# Autodesk Inventor assembly: Mechanism Platform
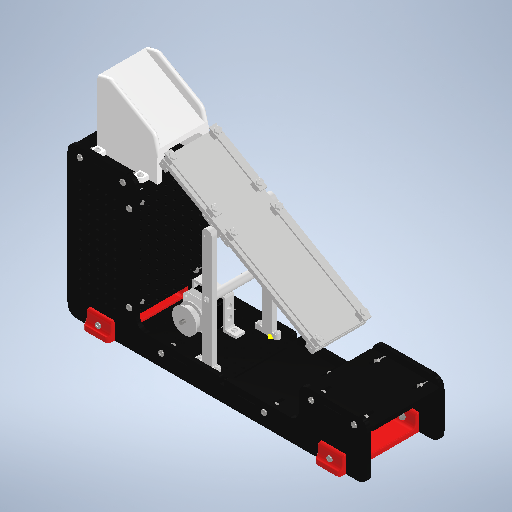
[picture p0: Inventor's stored thumbnail of the model, 512x512]
Saved by Autodesk Inventor 2025 (Build 290162000, 162)
## iProperties
Manager: Yassa Basem
Company: ENG 1P13
Created: 2024-06-07
Part Number: Mechanism Platform
Document SubType Name: Assembly
Designer: Alex Forbes
Checked By: Yassa Basem
Engineer: Alex Forbes
Author: A 1P13 IAI
Title: Mechanism Platform
## Documents named in this file (21)
- C:\Users\liaco\OneDrive\Documents\Graphics Labs\1P13 CAD Models\Design 2\Platform Assembly\1. Platform\Mechanism Platform.iam
- C:\Users\liaco\OneDrive\Documents\Graphics Labs\1P13 CAD Models\Design 2\Platform Assembly\1. Platform\Mounting Base Middle.ipt
- C:\Users\liaco\OneDrive\Documents\Graphics Labs\1P13 CAD Models\Design 2\Platform Assembly\1. Platform\Mounting Base Side.ipt
- C:\Users\liaco\OneDrive\Documents\Graphics Labs\1P13 CAD Models\Design 2\Platform Assembly\1. Platform\ANSI B 18.2.4.1 M - M4 x 0.7Style 1.ipt
- C:\Users\liaco\OneDrive\Documents\Graphics Labs\1P13 CAD Models\Design 2\Platform Assembly\1. Platform\Mounting Base Bottom.ipt
- C:\Users\liaco\OneDrive\Documents\Graphics Labs\1P13 CAD Models\Design 2\Platform Assembly\1. Platform\ANSI B18.6.7M - M4x0.7 x 20(4).ipt
- C:\Users\liaco\OneDrive\Documents\Graphics Labs\1P13 CAD Models\Design 2\Platform Assembly\1. Platform\Mounting Feet.ipt
- C:\Users\liaco\OneDrive\Documents\Graphics Labs\1P13 CAD Models\Design 2\Platform Assembly\1. Platform\Mounting Side Wall.ipt
- C:\Users\liaco\OneDrive\Documents\Graphics Labs\1P13 CAD Models\Design 2\Platform Assembly\1. Platform\Mounting Base Top.ipt
- C:\Users\liaco\OneDrive\Documents\Graphics Labs\1P13 CAD Models\Design 2\Top Ramp.ipt
- C:\Users\liaco\OneDrive\Documents\Graphics Labs\1P13 CAD Models\Design 2\Slide Strut.ipt
- C:\Users\liaco\OneDrive\Documents\Graphics Labs\1P13 CAD Models\Design 2\Slide Axle.ipt
- C:\Users\liaco\OneDrive\Documents\Graphics Labs\1P13 CAD Models\Design 2\Rotary Actuator Assembly\4. Rotary Actuator\Stepper Motor NEMA 17.iam
- C:\Users\liaco\OneDrive\Documents\Graphics Labs\1P13 CAD Models\Design 2\Rotary Actuator Mount.ipt
- C:\Users\liaco\OneDrive\Documents\Graphics Labs\1P13 CAD Models\Design 2\Pulley.ipt
- C:\Users\liaco\OneDrive\Documents\Graphics Labs\1P13 CAD Models\Design 2\Slide Assembly V2.iam
- C:\Users\liaco\OneDrive\Documents\Graphics Labs\1P13 CAD Models\Design 2\2. Plate Fasteners\M4 x 16mm Machine Screw.ipt
- C:\Users\liaco\OneDrive\Documents\Graphics Labs\1P13 CAD Models\Design 2\support pole.ipt
- C:\Users\liaco\OneDrive\Documents\Graphics Labs\1P13 CAD Models\Design 2\91251A198_Black-Oxide Alloy Steel Socket Head Screw\91251A198_Black-Oxide Alloy Steel Socket Head Screw.ipt
- C:\Users\liaco\OneDrive\Documents\Graphics Labs\1P13 CAD Models\Design 2\2. Plate Fasteners\M4 Nut.ipt
- C:\Users\liaco\OneDrive\Documents\Graphics Labs\1P13 CAD Models\Design 2\90480A009_Low-Strength Steel Hex Nut\90480A009_Low-Strength Steel Hex Nut.ipt
## Components (95 placed, 20 different names)
1. Top Ramp:1 — Mate:200, Mate:201, Mate:202, Mate:240, Mate:241, Mate:242, Mate:243, Mate:244, Mate:245, Mate:246, Mate:247
2. Slide Axle:1 — Angle:11, Mate:224, Mate:234, Flush:5, Angle:13
3. Stepper Motor NEMA 17:1 [sub-assembly] — Flush:4, Mate:265, Mate:266, Mate:267, Flush:6, Mate:272
4. Rotary Actuator Mount:1 — Mate:221, Flush:4, Mate:222, Mate:223, Mate:248, Mate:249, Mate:250, Mate:251, Mate:265, Mate:266
5. Pulley:1 — Mate:267, Flush:6, Mate:272
6. Slide Assembly V2:1 [sub-assembly] — Mate:224, Mate:235, Angle:12, Mate:273, Mate:274, Mate:275, Mate:276, Mate:277, Mate:278, Mate:279, Mate:280, Mate:281, Mate:282, Mate:283, Mate:284, Mate:285, Mate:286, Mate:287, Mate:288, Mate:300, Mate:303, Mate:304, Mate:306, Mate:311, Mate:312, Mate:313, Mate:314
7. Slide Strut:2 — Mate:227, Mate:234, Mate:235, Mate:236, Mate:237, Mate:252, Mate:253, Mate:258, Mate:259, Mate:260, Mate:262, Flush:5, Mate:268, Mate:271
8. Slide Strut:3 — Mate:231, Mate:238, Mate:239, Mate:254, Mate:255, Mate:256, Mate:257, Mate:263, Mate:264, Mate:269, Mate:270
9. support pole:1 — Mate:260, Mate:262, Mate:263, Mate:264, Angle:14
10. Mounting Side Wall:1 — Insert:1, Angle:1, Insert:2, Mate:1, Mate:2, Mate:3, Mate:4, Flush:1, Flush:2, Mate:5, Angle:3, Mate:6, Mate:7, Mate:8, Mate:9, Mate:50, Mate:51, Mate:52, Mate:53, Mate:109, Mate:110, Mate:111, Mate:129, Mate:130, Mate:131, Mate:133, Mate:134, Mate:135, Mate:145, Mate:146, Mate:147, Mate:149, Mate:150, Mate:151, Mate:157, Mate:158, Mate:159, Mate:169, Mate:170, Mate:171, Mate:173, Mate:174, Mate:175, Angle:13
11. Mounting Side Wall:2 — Mate:4, Flush:1, Flush:2, Mate:117, Mate:118, Mate:119, Mate:121, Mate:122, Mate:123, Mate:125, Mate:126, Mate:127, Mate:137, Mate:138, Mate:139, Mate:141, Mate:142, Mate:143, Mate:153, Mate:154, Mate:155, Mate:161, Mate:162, Mate:163, Mate:165, Mate:166, Mate:167
12. Mounting Base Top:1 — Mate:1, Mate:8, Mate:9, Mate:112, Mate:120, Mate:124, Mate:176, Angle:6, Angle:7, Mate:200, Mate:201, Mate:202
13. Mounting Base Middle:1 — Mate:2, Mate:52, Mate:53, Mate:144, Mate:148, Mate:152, Mate:156, Mate:221, Mate:222, Mate:223, Mate:227, Mate:231, Mate:236, Mate:237, Mate:238, Mate:239, Angle:12
14. Mounting Base Bottom:1 — Mate:3, Mate:50, Mate:51, Mate:160, Mate:164, Mate:168, Mate:172, Angle:4, Angle:5
15. Mounting Base Side:1 — Mate:5, Angle:3, Mate:6, Mate:7, Mate:128, Mate:132, Mate:136, Mate:140
16. Mounting Feet:1 — Insert:1, Angle:1, Angle:2, Mate:177, Mate:178, Mate:179, Mate:180, Mate:181, Mate:182, Mate:183, Mate:184
17. Mounting Feet:2 — Insert:2, Angle:2, Mate:185, Mate:186, Mate:187, Mate:188, Mate:189, Mate:190, Mate:191, Mate:192
18. Cross Recessed Pan Head Machine Screw - Type I - Metric M4x0.7 x 20:1 — Mate:173, Mate:174
19. Hex Nut Metric M4 x 0.7:1 — Mate:175, Mate:176
20. Cross Recessed Pan Head Machine Screw - Type I - Metric M4x0.7 x 20:7 — Mate:129, Mate:130
21. Hex Nut Metric M4 x 0.7:3 — Mate:131, Mate:132
22. Cross Recessed Pan Head Machine Screw - Type I - Metric M4x0.7 x 20:8 — Mate:133, Mate:134
23. Hex Nut Metric M4 x 0.7:5 — Mate:135, Mate:136
24. Cross Recessed Pan Head Machine Screw - Type I - Metric M4x0.7 x 20:5 — Mate:121, Mate:122
25. Hex Nut Metric M4 x 0.7:6 — Mate:123, Mate:124
26. Cross Recessed Pan Head Machine Screw - Type I - Metric M4x0.7 x 20:4 — Mate:117, Mate:118
27. Hex Nut Metric M4 x 0.7:7 — Mate:119, Mate:120
28. Cross Recessed Pan Head Machine Screw - Type I - Metric M4x0.7 x 20:6 — Mate:125, Mate:126
29. Hex Nut Metric M4 x 0.7:8 — Mate:127, Mate:128
30. Cross Recessed Pan Head Machine Screw - Type I - Metric M4x0.7 x 20:3 — Mate:137, Mate:138
31. Hex Nut Metric M4 x 0.7:10 — Mate:139, Mate:140
32. Cross Recessed Pan Head Machine Screw - Type I - Metric M4x0.7 x 20:10 — Mate:145, Mate:146
33. Hex Nut Metric M4 x 0.7:11 — Mate:147, Mate:148
34. Cross Recessed Pan Head Machine Screw - Type I - Metric M4x0.7 x 20:11 — Mate:149, Mate:150
35. Hex Nut Metric M4 x 0.7:13 — Mate:151, Mate:152
36. Cross Recessed Pan Head Machine Screw - Type I - Metric M4x0.7 x 20:9 — Mate:141, Mate:142
37. Hex Nut Metric M4 x 0.7:14 — Mate:143, Mate:144
38. Cross Recessed Pan Head Machine Screw - Type I - Metric M4x0.7 x 20:12 — Mate:153, Mate:154
39. Hex Nut Metric M4 x 0.7:16 — Mate:155, Mate:156
40. Cross Recessed Pan Head Machine Screw - Type I - Metric M4x0.7 x 20:13 — Mate:157, Mate:158
41. Hex Nut Metric M4 x 0.7:17 — Mate:159, Mate:160
42. Cross Recessed Pan Head Machine Screw - Type I - Metric M4x0.7 x 20:16 — Mate:169, Mate:170
43. Hex Nut Metric M4 x 0.7:18 — Mate:171, Mate:172
44. Cross Recessed Pan Head Machine Screw - Type I - Metric M4x0.7 x 20:14 — Mate:161, Mate:162
45. Hex Nut Metric M4 x 0.7:19 — Mate:163, Mate:164
46. Cross Recessed Pan Head Machine Screw - Type I - Metric M4x0.7 x 20:15 — Mate:165, Mate:166
47. Hex Nut Metric M4 x 0.7:20 — Mate:167, Mate:168
48. Cross Recessed Pan Head Machine Screw - Type I - Metric M4x0.7 x 20:2 — Mate:109, Mate:110
49. Hex Nut Metric M4 x 0.7:21 — Mate:111, Mate:112
50. Cross Recessed Pan Head Machine Screw - Type I - Metric M4x0.7 x 20:17 — Mate:177, Mate:178
51. Hex Nut Metric M4 x 0.7:22 — Mate:179, Mate:180, Angle:6
52. Cross Recessed Pan Head Machine Screw - Type I - Metric M4x0.7 x 20:18 — Mate:181, Mate:182
53. Hex Nut Metric M4 x 0.7:23 — Mate:183, Mate:184, Angle:7
54. Cross Recessed Pan Head Machine Screw - Type I - Metric M4x0.7 x 20:19 — Mate:185, Mate:186
55. Hex Nut Metric M4 x 0.7:24 — Mate:187, Mate:188, Angle:5
56. Cross Recessed Pan Head Machine Screw - Type I - Metric M4x0.7 x 20:20 — Mate:189, Mate:190
57. Hex Nut Metric M4 x 0.7:25 — Mate:191, Mate:192, Angle:4
58. 90480A009_Low-Strength Steel Hex Nut:8 — Mate:309, Mate:312
59. 90480A009_Low-Strength Steel Hex Nut:7 — Mate:310, Mate:311
60. 90480A009_Low-Strength Steel Hex Nut:6 — Mate:308, Mate:313
61. 90480A009_Low-Strength Steel Hex Nut:5 — Mate:307, Mate:314
62. 90480A009_Low-Strength Steel Hex Nut:4 — Mate:301, Mate:303
63. 90480A009_Low-Strength Steel Hex Nut:3 — Mate:302, Mate:304
64. 90480A009_Low-Strength Steel Hex Nut:2 — Mate:299, Mate:300
65. 90480A009_Low-Strength Steel Hex Nut:1 — Mate:305, Mate:306
66. M4 Nut:10 — Flush:8, Mate:290
67. M4 Nut:9 — Flush:7, Mate:289
68. M4 Nut:8 — Flush:9, Mate:291
69. M4 Nut:7 — Flush:11, Mate:293
70. M4 Nut:6 — Flush:10, Mate:292
71. M4 Nut:5 — Mate:294, Flush:12
72. M4 Nut:4 — Flush:13, Mate:295
73. M4 Nut:3 — Mate:298, Flush:16
74. M4 Nut:2 — Mate:296, Flush:14
75. M4 Nut:1 — Mate:297, Flush:15
76. 91251A198_Black-Oxide Alloy Steel Socket Head Screw:1 — Mate:273, Mate:277, Mate:299
77. 91251A198_Black-Oxide Alloy Steel Socket Head Screw:2 — Mate:276, Mate:280, Mate:305
78. 91251A198_Black-Oxide Alloy Steel Socket Head Screw:3 — Mate:274, Mate:278, Mate:301
79. 91251A198_Black-Oxide Alloy Steel Socket Head Screw:4 — Mate:275, Mate:279, Mate:302
80. 91251A198_Black-Oxide Alloy Steel Socket Head Screw:5 — Mate:284, Mate:288, Mate:307
81. 91251A198_Black-Oxide Alloy Steel Socket Head Screw:6 — Mate:283, Mate:287, Mate:308
82. 91251A198_Black-Oxide Alloy Steel Socket Head Screw:7 — Mate:282, Mate:286, Mate:309
83. 91251A198_Black-Oxide Alloy Steel Socket Head Screw:8 — Mate:281, Mate:285, Mate:310
84. M4 x 16mm Machine Screw:13 — Mate:269, Mate:270
85. M4 x 16mm Machine Screw:12 — Mate:268, Mate:271
86. M4 x 16mm Machine Screw:10 — Mate:253, Mate:259, Mate:297, Flush:15
87. M4 x 16mm Machine Screw:9 — Mate:254, Mate:257, Flush:13, Mate:295
88. M4 x 16mm Machine Screw:8 — Mate:252, Mate:258, Mate:298, Flush:16
89. M4 x 16mm Machine Screw:7 — Mate:255, Mate:256, Mate:296, Flush:14
90. M4 x 16mm Machine Screw:5 — Mate:243, Mate:245, Flush:10, Mate:292
91. M4 x 16mm Machine Screw:6 — Mate:242, Mate:244, Flush:9, Mate:291
92. M4 x 16mm Machine Screw:4 — Mate:240, Mate:247, Flush:7, Flush:8, Mate:290
93. M4 x 16mm Machine Screw:3 — Mate:241, Mate:246, Mate:289
94. M4 x 16mm Machine Screw:2 — Mate:248, Mate:250, Mate:294, Flush:12
95. M4 x 16mm Machine Screw:1 — Mate:249, Mate:251, Flush:11, Mate:293
## Relationships (210: Mate 182, Flush 15, Angle 11, Insert 2)
- Insert:1: Mounting Side Wall:1 ↔ Mounting Feet:1
- Angle:1 (0 deg): Mounting Side Wall:1 ↔ Mounting Feet:1
- Insert:2: Mounting Side Wall:1 ↔ Mounting Feet:2
- Angle:2 (0 deg): Mounting Feet:1 ↔ Mounting Feet:2
- Mate:1: Mounting Side Wall:1 ↔ Mounting Base Top:1
- Mate:2: Mounting Side Wall:1 ↔ Mounting Base Middle:1
- Mate:3: Mounting Side Wall:1 ↔ Mounting Base Bottom:1
- Mate:4 (102.3 mm): Mounting Side Wall:1 ↔ Mounting Side Wall:2
- Flush:1: Mounting Side Wall:1 ↔ Mounting Side Wall:2
- Flush:2: Mounting Side Wall:1 ↔ Mounting Side Wall:2
- Mate:5: Mounting Side Wall:1 ↔ Mounting Base Side:1
- Angle:3 (0 deg): Mounting Side Wall:1 ↔ Mounting Base Side:1
- Mate:6: Mounting Side Wall:1 ↔ Mounting Base Side:1
- Mate:7: Mounting Side Wall:1 ↔ Mounting Base Side:1
- Mate:8: Mounting Side Wall:1 ↔ Mounting Base Top:1
- Mate:9: Mounting Side Wall:1 ↔ Mounting Base Top:1
- Mate:50: Mounting Side Wall:1 ↔ Mounting Base Bottom:1
- Mate:51: Mounting Side Wall:1 ↔ Mounting Base Bottom:1
- Mate:52: Mounting Side Wall:1 ↔ Mounting Base Middle:1
- Mate:53: Mounting Side Wall:1 ↔ Mounting Base Middle:1
- Mate:109: Mounting Side Wall:1 ↔ Cross Recessed Pan Head Machine Screw - Type I - Metric M4x0.7 x 20:2
- Mate:110: Mounting Side Wall:1 ↔ Cross Recessed Pan Head Machine Screw - Type I - Metric M4x0.7 x 20:2
- Mate:111: Mounting Side Wall:1 ↔ Hex Nut Metric M4 x 0.7:21
- Mate:112: Mounting Base Top:1 ↔ Hex Nut Metric M4 x 0.7:21
- Mate:117: Mounting Side Wall:2 ↔ Cross Recessed Pan Head Machine Screw - Type I - Metric M4x0.7 x 20:4
- Mate:118: Mounting Side Wall:2 ↔ Cross Recessed Pan Head Machine Screw - Type I - Metric M4x0.7 x 20:4
- Mate:119: Mounting Side Wall:2 ↔ Hex Nut Metric M4 x 0.7:7
- Mate:120: Mounting Base Top:1 ↔ Hex Nut Metric M4 x 0.7:7
- Mate:121: Mounting Side Wall:2 ↔ Cross Recessed Pan Head Machine Screw - Type I - Metric M4x0.7 x 20:5
- Mate:122: Mounting Side Wall:2 ↔ Cross Recessed Pan Head Machine Screw - Type I - Metric M4x0.7 x 20:5
- Mate:123: Mounting Side Wall:2 ↔ Hex Nut Metric M4 x 0.7:6
- Mate:124: Mounting Base Top:1 ↔ Hex Nut Metric M4 x 0.7:6
- Mate:125: Mounting Side Wall:2 ↔ Cross Recessed Pan Head Machine Screw - Type I - Metric M4x0.7 x 20:6
- Mate:126: Mounting Side Wall:2 ↔ Cross Recessed Pan Head Machine Screw - Type I - Metric M4x0.7 x 20:6
- Mate:127: Mounting Side Wall:2 ↔ Hex Nut Metric M4 x 0.7:8
- Mate:128: Mounting Base Side:1 ↔ Hex Nut Metric M4 x 0.7:8
- Mate:129: Mounting Side Wall:1 ↔ Cross Recessed Pan Head Machine Screw - Type I - Metric M4x0.7 x 20:7
- Mate:130: Mounting Side Wall:1 ↔ Cross Recessed Pan Head Machine Screw - Type I - Metric M4x0.7 x 20:7
- Mate:131: Mounting Side Wall:1 ↔ Hex Nut Metric M4 x 0.7:3
- Mate:132: Mounting Base Side:1 ↔ Hex Nut Metric M4 x 0.7:3
- Mate:133: Mounting Side Wall:1 ↔ Cross Recessed Pan Head Machine Screw - Type I - Metric M4x0.7 x 20:8
- Mate:134: Mounting Side Wall:1 ↔ Cross Recessed Pan Head Machine Screw - Type I - Metric M4x0.7 x 20:8
- Mate:135: Mounting Side Wall:1 ↔ Hex Nut Metric M4 x 0.7:5
- Mate:136: Mounting Base Side:1 ↔ Hex Nut Metric M4 x 0.7:5
- Mate:137: Mounting Side Wall:2 ↔ Cross Recessed Pan Head Machine Screw - Type I - Metric M4x0.7 x 20:3
- Mate:138: Mounting Side Wall:2 ↔ Cross Recessed Pan Head Machine Screw - Type I - Metric M4x0.7 x 20:3
- Mate:139: Mounting Side Wall:2 ↔ Hex Nut Metric M4 x 0.7:10
- Mate:140: Mounting Base Side:1 ↔ Hex Nut Metric M4 x 0.7:10
- Mate:141: Mounting Side Wall:2 ↔ Cross Recessed Pan Head Machine Screw - Type I - Metric M4x0.7 x 20:9
- Mate:142: Mounting Side Wall:2 ↔ Cross Recessed Pan Head Machine Screw - Type I - Metric M4x0.7 x 20:9
- Mate:143: Mounting Side Wall:2 ↔ Hex Nut Metric M4 x 0.7:14
- Mate:144: Mounting Base Middle:1 ↔ Hex Nut Metric M4 x 0.7:14
- Mate:145: Mounting Side Wall:1 ↔ Cross Recessed Pan Head Machine Screw - Type I - Metric M4x0.7 x 20:10
- Mate:146: Mounting Side Wall:1 ↔ Cross Recessed Pan Head Machine Screw - Type I - Metric M4x0.7 x 20:10
- Mate:147: Mounting Side Wall:1 ↔ Hex Nut Metric M4 x 0.7:11
- Mate:148: Mounting Base Middle:1 ↔ Hex Nut Metric M4 x 0.7:11
- Mate:149: Mounting Side Wall:1 ↔ Cross Recessed Pan Head Machine Screw - Type I - Metric M4x0.7 x 20:11
- Mate:150: Mounting Side Wall:1 ↔ Cross Recessed Pan Head Machine Screw - Type I - Metric M4x0.7 x 20:11
- Mate:151: Mounting Side Wall:1 ↔ Hex Nut Metric M4 x 0.7:13
- Mate:152: Mounting Base Middle:1 ↔ Hex Nut Metric M4 x 0.7:13
- Mate:153: Mounting Side Wall:2 ↔ Cross Recessed Pan Head Machine Screw - Type I - Metric M4x0.7 x 20:12
- Mate:154: Mounting Side Wall:2 ↔ Cross Recessed Pan Head Machine Screw - Type I - Metric M4x0.7 x 20:12
- Mate:155: Mounting Side Wall:2 ↔ Hex Nut Metric M4 x 0.7:16
- Mate:156: Mounting Base Middle:1 ↔ Hex Nut Metric M4 x 0.7:16
- Mate:157: Mounting Side Wall:1 ↔ Cross Recessed Pan Head Machine Screw - Type I - Metric M4x0.7 x 20:13
- Mate:158: Mounting Side Wall:1 ↔ Cross Recessed Pan Head Machine Screw - Type I - Metric M4x0.7 x 20:13
- Mate:159: Mounting Side Wall:1 ↔ Hex Nut Metric M4 x 0.7:17
- Mate:160: Mounting Base Bottom:1 ↔ Hex Nut Metric M4 x 0.7:17
- Mate:161: Mounting Side Wall:2 ↔ Cross Recessed Pan Head Machine Screw - Type I - Metric M4x0.7 x 20:14
- Mate:162: Mounting Side Wall:2 ↔ Cross Recessed Pan Head Machine Screw - Type I - Metric M4x0.7 x 20:14
- Mate:163: Mounting Side Wall:2 ↔ Hex Nut Metric M4 x 0.7:19
- Mate:164: Mounting Base Bottom:1 ↔ Hex Nut Metric M4 x 0.7:19
- Mate:165: Mounting Side Wall:2 ↔ Cross Recessed Pan Head Machine Screw - Type I - Metric M4x0.7 x 20:15
- Mate:166: Mounting Side Wall:2 ↔ Cross Recessed Pan Head Machine Screw - Type I - Metric M4x0.7 x 20:15
- Mate:167: Mounting Side Wall:2 ↔ Hex Nut Metric M4 x 0.7:20
- Mate:168: Mounting Base Bottom:1 ↔ Hex Nut Metric M4 x 0.7:20
- Mate:169: Mounting Side Wall:1 ↔ Cross Recessed Pan Head Machine Screw - Type I - Metric M4x0.7 x 20:16
- Mate:170: Mounting Side Wall:1 ↔ Cross Recessed Pan Head Machine Screw - Type I - Metric M4x0.7 x 20:16
- Mate:171: Mounting Side Wall:1 ↔ Hex Nut Metric M4 x 0.7:18
- Mate:172: Mounting Base Bottom:1 ↔ Hex Nut Metric M4 x 0.7:18
- Mate:173: Mounting Side Wall:1 ↔ Cross Recessed Pan Head Machine Screw - Type I - Metric M4x0.7 x 20:1
- Mate:174: Mounting Side Wall:1 ↔ Cross Recessed Pan Head Machine Screw - Type I - Metric M4x0.7 x 20:1
- Mate:175: Mounting Side Wall:1 ↔ Hex Nut Metric M4 x 0.7:1
- Mate:176: Mounting Base Top:1 ↔ Hex Nut Metric M4 x 0.7:1
- Mate:177: Mounting Feet:1 ↔ Cross Recessed Pan Head Machine Screw - Type I - Metric M4x0.7 x 20:17
- Mate:178: Mounting Feet:1 ↔ Cross Recessed Pan Head Machine Screw - Type I - Metric M4x0.7 x 20:17
- Mate:179: Mounting Feet:1 ↔ Hex Nut Metric M4 x 0.7:22
- Mate:180: Mounting Feet:1 ↔ Hex Nut Metric M4 x 0.7:22
- Mate:181: Mounting Feet:1 ↔ Cross Recessed Pan Head Machine Screw - Type I - Metric M4x0.7 x 20:18
- Mate:182: Mounting Feet:1 ↔ Cross Recessed Pan Head Machine Screw - Type I - Metric M4x0.7 x 20:18
- Mate:183: Mounting Feet:1 ↔ Hex Nut Metric M4 x 0.7:23
- Mate:184: Mounting Feet:1 ↔ Hex Nut Metric M4 x 0.7:23
- Mate:185: Mounting Feet:2 ↔ Cross Recessed Pan Head Machine Screw - Type I - Metric M4x0.7 x 20:19
- Mate:186: Mounting Feet:2 ↔ Cross Recessed Pan Head Machine Screw - Type I - Metric M4x0.7 x 20:19
- Mate:187: Mounting Feet:2 ↔ Hex Nut Metric M4 x 0.7:24
- Mate:188: Mounting Feet:2 ↔ Hex Nut Metric M4 x 0.7:24
- Mate:189: Mounting Feet:2 ↔ Cross Recessed Pan Head Machine Screw - Type I - Metric M4x0.7 x 20:20
- Mate:190: Mounting Feet:2 ↔ Cross Recessed Pan Head Machine Screw - Type I - Metric M4x0.7 x 20:20
- Mate:191: Mounting Feet:2 ↔ Hex Nut Metric M4 x 0.7:25
- Mate:192: Mounting Feet:2 ↔ Hex Nut Metric M4 x 0.7:25
- Angle:4 (0 deg): Mounting Base Bottom:1 ↔ Hex Nut Metric M4 x 0.7:25
- Angle:5 (0 deg): Mounting Base Bottom:1 ↔ Hex Nut Metric M4 x 0.7:24
- Angle:6 (0 deg): Mounting Base Top:1 ↔ Hex Nut Metric M4 x 0.7:22
- Angle:7 (0 deg): Mounting Base Top:1 ↔ Hex Nut Metric M4 x 0.7:23
- Mate:200: Top Ramp:1 ↔ Mounting Base Top:1
- Mate:201: Top Ramp:1 ↔ Mounting Base Top:1
- Mate:202: Top Ramp:1 ↔ Mounting Base Top:1
- Mate:221: Rotary Actuator Mount:1 ↔ Mounting Base Middle:1
- Flush:4: Stepper Motor NEMA 17:1 ↔ Rotary Actuator Mount:1
- Mate:222: Rotary Actuator Mount:1 ↔ Mounting Base Middle:1
- Mate:223: Rotary Actuator Mount:1 ↔ Mounting Base Middle:1
- Angle:11 (0 deg): Slide Axle:1
- Mate:224: Slide Axle:1 ↔ Slide Assembly V2:1
- Mate:227: Slide Strut:2 ↔ Mounting Base Middle:1
- Mate:231: Slide Strut:3 ↔ Mounting Base Middle:1
- Mate:234: Slide Axle:1 ↔ Slide Strut:2
- Mate:235 (0.5 mm): Slide Assembly V2:1 ↔ Slide Strut:2
- Mate:236: Slide Strut:2 ↔ Mounting Base Middle:1
- Mate:237: Slide Strut:2 ↔ Mounting Base Middle:1
- Mate:238: Slide Strut:3 ↔ Mounting Base Middle:1
- Mate:239: Slide Strut:3 ↔ Mounting Base Middle:1
- Mate:240: Top Ramp:1 ↔ M4 x 16mm Machine Screw:4
- Mate:241: Top Ramp:1 ↔ M4 x 16mm Machine Screw:3
- Mate:242: Top Ramp:1 ↔ M4 x 16mm Machine Screw:6
- Mate:243: Top Ramp:1 ↔ M4 x 16mm Machine Screw:5
- Mate:244: Top Ramp:1 ↔ M4 x 16mm Machine Screw:6
- Mate:245: Top Ramp:1 ↔ M4 x 16mm Machine Screw:5
- Mate:246: Top Ramp:1 ↔ M4 x 16mm Machine Screw:3
- Mate:247: Top Ramp:1 ↔ M4 x 16mm Machine Screw:4
- Mate:248: Rotary Actuator Mount:1 ↔ M4 x 16mm Machine Screw:2
- Mate:249: Rotary Actuator Mount:1 ↔ M4 x 16mm Machine Screw:1
- Mate:250: Rotary Actuator Mount:1 ↔ M4 x 16mm Machine Screw:2
- Mate:251: Rotary Actuator Mount:1 ↔ M4 x 16mm Machine Screw:1
- Mate:252: Slide Strut:2 ↔ M4 x 16mm Machine Screw:8
- Mate:253: Slide Strut:2 ↔ M4 x 16mm Machine Screw:10
- Mate:254: Slide Strut:3 ↔ M4 x 16mm Machine Screw:9
- Mate:255: Slide Strut:3 ↔ M4 x 16mm Machine Screw:7
- Mate:256: Slide Strut:3 ↔ M4 x 16mm Machine Screw:7
- Mate:257: Slide Strut:3 ↔ M4 x 16mm Machine Screw:9
- Mate:258: Slide Strut:2 ↔ M4 x 16mm Machine Screw:8
- Mate:259: Slide Strut:2 ↔ M4 x 16mm Machine Screw:10
- Mate:260: Slide Strut:2 ↔ support pole:1
- Mate:262: Slide Strut:2 ↔ support pole:1
- Mate:263: Slide Strut:3 ↔ support pole:1
- Mate:264: Slide Strut:3 ↔ support pole:1
- Angle:12 (270 deg): Slide Assembly V2:1 ↔ Mounting Base Middle:1
- Flush:5: Slide Axle:1 ↔ Slide Strut:2
- Angle:13 (0 deg): Slide Axle:1 ↔ Mounting Side Wall:1
- Mate:265: Stepper Motor NEMA 17:1 ↔ Rotary Actuator Mount:1
- Mate:266: Stepper Motor NEMA 17:1 ↔ Rotary Actuator Mount:1
- Mate:267: Stepper Motor NEMA 17:1 ↔ Pulley:1
- Flush:6 (6 mm): Stepper Motor NEMA 17:1 ↔ Pulley:1
- Mate:268: Slide Strut:2 ↔ M4 x 16mm Machine Screw:12
- Mate:269: Slide Strut:3 ↔ M4 x 16mm Machine Screw:13
- Mate:270: Slide Strut:3 ↔ M4 x 16mm Machine Screw:13
- Mate:271: Slide Strut:2 ↔ M4 x 16mm Machine Screw:12
- Mate:272: Stepper Motor NEMA 17:1 ↔ Pulley:1
- Angle:14 (0 deg): support pole:1
- Mate:273: Slide Assembly V2:1 ↔ 91251A198_Black-Oxide Alloy Steel Socket Head Screw:1
- Mate:274: Slide Assembly V2:1 ↔ 91251A198_Black-Oxide Alloy Steel Socket Head Screw:3
- Mate:275: Slide Assembly V2:1 ↔ 91251A198_Black-Oxide Alloy Steel Socket Head Screw:4
- Mate:276: Slide Assembly V2:1 ↔ 91251A198_Black-Oxide Alloy Steel Socket Head Screw:2
- Mate:277: Slide Assembly V2:1 ↔ 91251A198_Black-Oxide Alloy Steel Socket Head Screw:1
- Mate:278: Slide Assembly V2:1 ↔ 91251A198_Black-Oxide Alloy Steel Socket Head Screw:3
- Mate:279: Slide Assembly V2:1 ↔ 91251A198_Black-Oxide Alloy Steel Socket Head Screw:4
- Mate:280: Slide Assembly V2:1 ↔ 91251A198_Black-Oxide Alloy Steel Socket Head Screw:2
- Mate:281: Slide Assembly V2:1 ↔ 91251A198_Black-Oxide Alloy Steel Socket Head Screw:8
- Mate:282: Slide Assembly V2:1 ↔ 91251A198_Black-Oxide Alloy Steel Socket Head Screw:7
- Mate:283: Slide Assembly V2:1 ↔ 91251A198_Black-Oxide Alloy Steel Socket Head Screw:6
- Mate:284: Slide Assembly V2:1 ↔ 91251A198_Black-Oxide Alloy Steel Socket Head Screw:5
- Mate:285: Slide Assembly V2:1 ↔ 91251A198_Black-Oxide Alloy Steel Socket Head Screw:8
- Mate:286: Slide Assembly V2:1 ↔ 91251A198_Black-Oxide Alloy Steel Socket Head Screw:7
- Mate:287: Slide Assembly V2:1 ↔ 91251A198_Black-Oxide Alloy Steel Socket Head Screw:6
- Mate:288: Slide Assembly V2:1 ↔ 91251A198_Black-Oxide Alloy Steel Socket Head Screw:5
- Flush:7: M4 Nut:9 ↔ M4 x 16mm Machine Screw:4
- Mate:289: M4 Nut:9 ↔ M4 x 16mm Machine Screw:3
- Flush:8: M4 Nut:10 ↔ M4 x 16mm Machine Screw:4
- Mate:290: M4 Nut:10 ↔ M4 x 16mm Machine Screw:4
- Flush:9: M4 Nut:8 ↔ M4 x 16mm Machine Screw:6
- Mate:291: M4 Nut:8 ↔ M4 x 16mm Machine Screw:6
- Flush:10: M4 Nut:6 ↔ M4 x 16mm Machine Screw:5
- Mate:292: M4 Nut:6 ↔ M4 x 16mm Machine Screw:5
- Flush:11: M4 Nut:7 ↔ M4 x 16mm Machine Screw:1
- Mate:293: M4 Nut:7 ↔ M4 x 16mm Machine Screw:1
- Mate:294: M4 Nut:5 ↔ M4 x 16mm Machine Screw:2
- Flush:12: M4 Nut:5 ↔ M4 x 16mm Machine Screw:2
- Flush:13: M4 Nut:4 ↔ M4 x 16mm Machine Screw:9
- Mate:295: M4 Nut:4 ↔ M4 x 16mm Machine Screw:9
- Mate:296: M4 Nut:2 ↔ M4 x 16mm Machine Screw:7
- Flush:14: M4 Nut:2 ↔ M4 x 16mm Machine Screw:7
- Mate:297: M4 Nut:1 ↔ M4 x 16mm Machine Screw:10
- Flush:15: M4 Nut:1 ↔ M4 x 16mm Machine Screw:10
- Mate:298: M4 Nut:3 ↔ M4 x 16mm Machine Screw:8
- Flush:16: M4 Nut:3 ↔ M4 x 16mm Machine Screw:8
- Mate:299: 90480A009_Low-Strength Steel Hex Nut:2 ↔ 91251A198_Black-Oxide Alloy Steel Socket Head Screw:1
- Mate:300: Slide Assembly V2:1 ↔ 90480A009_Low-Strength Steel Hex Nut:2
- Mate:301: 90480A009_Low-Strength Steel Hex Nut:4 ↔ 91251A198_Black-Oxide Alloy Steel Socket Head Screw:3
- Mate:302: 90480A009_Low-Strength Steel Hex Nut:3 ↔ 91251A198_Black-Oxide Alloy Steel Socket Head Screw:4
- Mate:303: Slide Assembly V2:1 ↔ 90480A009_Low-Strength Steel Hex Nut:4
- Mate:304: Slide Assembly V2:1 ↔ 90480A009_Low-Strength Steel Hex Nut:3
- Mate:305: 90480A009_Low-Strength Steel Hex Nut:1 ↔ 91251A198_Black-Oxide Alloy Steel Socket Head Screw:2
- Mate:306: Slide Assembly V2:1 ↔ 90480A009_Low-Strength Steel Hex Nut:1
- Mate:307: 90480A009_Low-Strength Steel Hex Nut:5 ↔ 91251A198_Black-Oxide Alloy Steel Socket Head Screw:5
- Mate:308: 90480A009_Low-Strength Steel Hex Nut:6 ↔ 91251A198_Black-Oxide Alloy Steel Socket Head Screw:6
- Mate:309: 90480A009_Low-Strength Steel Hex Nut:8 ↔ 91251A198_Black-Oxide Alloy Steel Socket Head Screw:7
- Mate:310: 90480A009_Low-Strength Steel Hex Nut:7 ↔ 91251A198_Black-Oxide Alloy Steel Socket Head Screw:8
- Mate:311: Slide Assembly V2:1 ↔ 90480A009_Low-Strength Steel Hex Nut:7
- Mate:312: Slide Assembly V2:1 ↔ 90480A009_Low-Strength Steel Hex Nut:8
- Mate:313: Slide Assembly V2:1 ↔ 90480A009_Low-Strength Steel Hex Nut:6
- Mate:314: Slide Assembly V2:1 ↔ 90480A009_Low-Strength Steel Hex Nut:5
